# Autodesk Inventor assembly: SC10
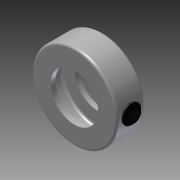
[picture p0: Inventor's stored thumbnail of the model, 180x180]
Saved by Autodesk Inventor 2014 (Build 180170000, 170)
## iProperties
Category: Miscellaneous
Company: Autodesk Inc.
Created: 2013-12-18
Part Number: SC10
Document SubType Name: Assembly
Designer: Autodesk Inc.
Catalog Web Link: http://www.triangleoshkosh.com/eng/products/oil-cups-shaft-collars/shaft-collars
Description: 5/8" ID 1.125 OD Set Screw Shaft Collar
Vendor: Traingle Manufacturing
Author: Autodesk Inc.
## Documents named in this file (3)
- D:\Data Folder\FIRST 2014\KOP Parts\Miscellaneous\MISC_ShaftCollar_SC10.iam
- D:\Data Folder\FIRST 2014\KOP Parts\Miscellaneous\Parts\MISC_ShaftCollar_SC10.ipt
- D:\Data Folder\FIRST 2014\KOP Parts\Miscellaneous\Parts\ANSI B18.3 - 1_4-20 UNC - 0.25(24).ipt
## Components (2 placed, 2 different names)
1. MISC_ShaftCollar_SC10:1 — Mate:1
2. Hexagon Socket Set Screw - Flat Point - Inch 1/4-20 UNC x 0.25:1 — Mate:1, Flush:1
## Relationships (2: Mate 1, Flush 1)
- Mate:1: MISC_ShaftCollar_SC10:1 ↔ Hexagon Socket Set Screw - Flat Point - Inch 1/4-20 UNC x 0.25:1
- Flush:1 (-15.24 mm): Hexagon Socket Set Screw - Flat Point - Inch 1/4-20 UNC x 0.25:1
